# Autodesk Inventor assembly: Pancake_Exit Assy_3 Lanes
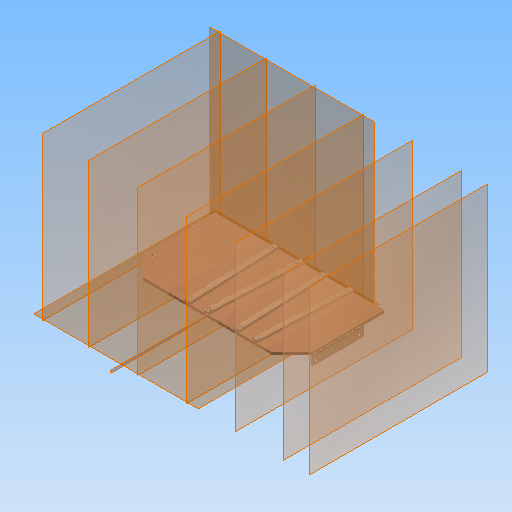
[picture p0: Inventor's stored thumbnail of the model, 512x512]
Saved by Autodesk Inventor 2018.1 (Build 221171000, 171)
## iProperties
Created: 2019-02-22
Part Number: Pancake_Exit Assy_3 Lanes
Document SubType Name: Assembly
Designer: James
Author: James
## Documents named in this file (7)
- C:\Users\admin\Desktop\Ball Sorting Machine\Ball-Sorting-Machine\Pancake Sort\Pancake - 3 Lanes\Pancake_Exit Assy_3 Lanes.iam
- C:\Users\admin\Desktop\Ball Sorting Machine\Ball-Sorting-Machine\Pancake Sort\Pancake_Angle Bracket 2.ipt
- C:\Users\admin\Desktop\Ball Sorting Machine\Ball-Sorting-Machine\Pancake Sort\Nyloc Nut - M4.ipt
- C:\Users\admin\Desktop\Ball Sorting Machine\Ball-Sorting-Machine\Pancake Sort\Socket Csk Screw - (A2) - M4 x  12.ipt
- C:\Users\admin\Desktop\Ball Sorting Machine\Ball-Sorting-Machine\Pancake Sort\Pancake_Exit Piece.ipt
- C:\Users\admin\Desktop\Ball Sorting Machine\Ball-Sorting-Machine\Pancake Sort\Socket Csk Screw - (A2) - M4 x  16.ipt
- C:\Users\admin\Desktop\Ball Sorting Machine\Ball-Sorting-Machine\Pancake Sort\Pancake - 3 Lanes\Pancake_Exit Board_3 Lanes.ipt
## Components (31 placed, 6 different names)
1. Pancake_Exit Board_3 Lanes:1 — Flush:1, Flush:2, Flush:3, Mate:1, Mate:2, Tangent:1, Tangent:2, Mate:5, Mate:6, Mate:7, Mate:8, Flush:5, Mate:21, Mate:24, Mate:25, Flush:9, Mate:29, Mate:30, Tangent:5, Tangent:6, Mate:33, Mate:34, Mate:36, Mate:40, Mate:42, Mate:50, Mate:51, Mate:52, Mate:53, Mate:54
2. Pancake_Angle Bracket 2:1 — Mate:6, Mate:7, Mate:8, Flush:5
3. Nyloc Nut - M4:1 — Mate:3, Flush:4, Mate:5
4. Socket Csk Screw - (A2) - M4 x  12:1 — Mate:1, Tangent:2, Mate:4
5. Nyloc Nut - M4:2 — Mate:4, Flush:4
6. Socket Csk Screw - (A2) - M4 x  12:2 — Mate:2, Tangent:1, Mate:3
7. Pancake_Angle Bracket 2:4 — Mate:21, Mate:24, Mate:25, Flush:9, Mate:32
8. Nyloc Nut - M4:7
9. Socket Csk Screw - (A2) - M4 x  12:7 — Mate:29, Tangent:6
10. Nyloc Nut - M4:8 — Mate:32
11. Socket Csk Screw - (A2) - M4 x  12:8 — Mate:30, Tangent:5
12. Pancake_Exit Piece:1 — Mate:33, Mate:34, Mate:36, Mate:37, Mate:39, Tangent:9, Tangent:10
13. Socket Csk Screw - (A2) - M4 x  16:5
14. Nyloc Nut - M4:13 — Mate:53
15. Socket Csk Screw - (A2) - M4 x  16:4
16. Nyloc Nut - M4:12 — Mate:54
17. Pancake_Exit Piece:2 — Mate:50, Mate:51, Mate:52
18. Socket Csk Screw - (A2) - M4 x  16:3 — Mate:39, Tangent:9, Mate:45
19. Nyloc Nut - M4:11 — Mate:42, Mate:45
20. Nyloc Nut - M4:9 — Mate:40, Mate:43
21. Socket Csk Screw - (A2) - M4 x  16:1 — Mate:37, Tangent:10, Mate:43
22. Pancake_Exit Piece:3
23. Socket Csk Screw - (A2) - M4 x  16:6
24. Nyloc Nut - M4:14
25. Socket Csk Screw - (A2) - M4 x  16:7
26. Nyloc Nut - M4:15
27. Pancake_Exit Piece:4
28. Socket Csk Screw - (A2) - M4 x  16:8
29. Nyloc Nut - M4:16
30. Nyloc Nut - M4:17
31. Socket Csk Screw - (A2) - M4 x  16:9
## Component patterns: (2 elements, first: Pancake_Exit Piece:1 + Socket Csk Screw - (A2) - M4 x  16:5 + Nyloc Nut - M4:13 + Socket Csk Screw - (A2) - M4 x  16:4 + Nyloc Nut - M4:12 + Pancake_Exit Piece:2 + Socket Csk Screw - (A2) - M4 x  16:3 + Nyloc Nut - M4:11 + Nyloc Nut - M4:9 + Socket Csk Screw - (A2) - M4 x  16:1)
## Relationships (49: Mate 34, Tangent 8, Flush 7)
- Flush:1: Pancake_Exit Board_3 Lanes:1
- Flush:2: Pancake_Exit Board_3 Lanes:1
- Flush:3: Pancake_Exit Board_3 Lanes:1
- Mate:1: Pancake_Exit Board_3 Lanes:1 ↔ Socket Csk Screw - (A2) - M4 x  12:1
- Mate:2: Pancake_Exit Board_3 Lanes:1 ↔ Socket Csk Screw - (A2) - M4 x  12:2
- Tangent:1: Pancake_Exit Board_3 Lanes:1 ↔ Socket Csk Screw - (A2) - M4 x  12:2
- Tangent:2: Pancake_Exit Board_3 Lanes:1 ↔ Socket Csk Screw - (A2) - M4 x  12:1
- Mate:3: Nyloc Nut - M4:1 ↔ Socket Csk Screw - (A2) - M4 x  12:2
- Mate:4: Socket Csk Screw - (A2) - M4 x  12:1 ↔ Nyloc Nut - M4:2
- Flush:4: Nyloc Nut - M4:1 ↔ Nyloc Nut - M4:2
- Mate:5 (3 mm): Pancake_Exit Board_3 Lanes:1 ↔ Nyloc Nut - M4:1
- Mate:6: Pancake_Exit Board_3 Lanes:1 ↔ Pancake_Angle Bracket 2:1
- Mate:7: Pancake_Exit Board_3 Lanes:1 ↔ Pancake_Angle Bracket 2:1
- Mate:8: Pancake_Exit Board_3 Lanes:1 ↔ Pancake_Angle Bracket 2:1
- Flush:5: Pancake_Exit Board_3 Lanes:1 ↔ Pancake_Angle Bracket 2:1
- [Mate]: Nyloc Nut - M4:7 ↔ Socket Csk Screw - (A2) - M4 x  12:8
- [Mate]: Socket Csk Screw - (A2) - M4 x  12:7 ↔ Nyloc Nut - M4:8
- [Flush]: Nyloc Nut - M4:7 ↔ Nyloc Nut - M4:8
- Mate:21: Pancake_Exit Board_3 Lanes:1 ↔ Pancake_Angle Bracket 2:4
- Mate:24: Pancake_Exit Board_3 Lanes:1 ↔ Pancake_Angle Bracket 2:4
- Mate:25: Pancake_Exit Board_3 Lanes:1 ↔ Pancake_Angle Bracket 2:4
- Flush:9: Pancake_Exit Board_3 Lanes:1 ↔ Pancake_Angle Bracket 2:4
- Mate:29: Pancake_Exit Board_3 Lanes:1 ↔ Socket Csk Screw - (A2) - M4 x  12:7
- Mate:30: Pancake_Exit Board_3 Lanes:1 ↔ Socket Csk Screw - (A2) - M4 x  12:8
- Tangent:5: Pancake_Exit Board_3 Lanes:1 ↔ Socket Csk Screw - (A2) - M4 x  12:8
- Tangent:6: Pancake_Exit Board_3 Lanes:1 ↔ Socket Csk Screw - (A2) - M4 x  12:7
- Mate:32: Pancake_Angle Bracket 2:4 ↔ Nyloc Nut - M4:8
- Mate:33: Pancake_Exit Board_3 Lanes:1 ↔ Pancake_Exit Piece:1
- Mate:34: Pancake_Exit Board_3 Lanes:1 ↔ Pancake_Exit Piece:1
- Mate:36: Pancake_Exit Board_3 Lanes:1 ↔ Pancake_Exit Piece:1
- Mate:37: Pancake_Exit Piece:1 ↔ Socket Csk Screw - (A2) - M4 x  16:1
- Mate:39: Pancake_Exit Piece:1 ↔ Socket Csk Screw - (A2) - M4 x  16:3
- Tangent:9: Pancake_Exit Piece:1 ↔ Socket Csk Screw - (A2) - M4 x  16:3
- Tangent:10: Pancake_Exit Piece:1 ↔ Socket Csk Screw - (A2) - M4 x  16:1
- Mate:40: Pancake_Exit Board_3 Lanes:1 ↔ Nyloc Nut - M4:9
- Mate:42: Pancake_Exit Board_3 Lanes:1 ↔ Nyloc Nut - M4:11
- Mate:43: Nyloc Nut - M4:9 ↔ Socket Csk Screw - (A2) - M4 x  16:1
- Mate:45: Socket Csk Screw - (A2) - M4 x  16:3 ↔ Nyloc Nut - M4:11
- [Mate]: Socket Csk Screw - (A2) - M4 x  16:4 ↔ Pancake_Exit Piece:2
- [Mate]: Socket Csk Screw - (A2) - M4 x  16:5 ↔ Pancake_Exit Piece:2
- [Tangent]: Socket Csk Screw - (A2) - M4 x  16:5 ↔ Pancake_Exit Piece:2
- [Tangent]: Socket Csk Screw - (A2) - M4 x  16:4 ↔ Pancake_Exit Piece:2
- [Mate]: Socket Csk Screw - (A2) - M4 x  16:4 ↔ Nyloc Nut - M4:12
- [Mate]: Socket Csk Screw - (A2) - M4 x  16:5 ↔ Nyloc Nut - M4:13
- Mate:50: Pancake_Exit Board_3 Lanes:1 ↔ Pancake_Exit Piece:2
- Mate:51: Pancake_Exit Board_3 Lanes:1 ↔ Pancake_Exit Piece:2
- Mate:52: Pancake_Exit Board_3 Lanes:1 ↔ Pancake_Exit Piece:2
- Mate:53: Pancake_Exit Board_3 Lanes:1 ↔ Nyloc Nut - M4:13
- Mate:54: Pancake_Exit Board_3 Lanes:1 ↔ Nyloc Nut - M4:12
## Named parameters: d21_d7 = 0 mm, d22_d8 = 0 mm, d23_d9 = 0 mm, d84_d56 = 0 mm, d85_d58 = 0 mm, d86_d59 = 0 mm, d87_d60 = 0 mm, d88_d65 = 0 mm, d89_d67 = 0 mm
